# Autodesk Inventor assembly: Robot_Triciclo_(assembled_fixed)
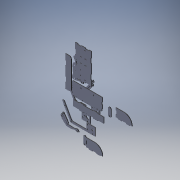
[picture p0: Inventor's stored thumbnail of the model, 180x180]
Saved by Autodesk Inventor 2019 (Build 230136000, 136)
## iProperties
Created: 2019-11-11
Part Number: Robot_Triciclo_(assembled_fixed)
Document SubType Name: Assembly
Designer: Domenico
Author: Domenico
Revision Number: ANY
## Documents named in this file (18)
- C:\Users\Domenico\Documents\Inventor\Mecanismos2\Robot_Triciclo_(assembled_fixed).iam
- C:\Users\Domenico\Documents\Inventor\Mecanismos2\Robot_Triciclo_(bike01).ipt
- C:\Users\Domenico\Documents\Inventor\Mecanismos2\Robot_Triciclo_(bike02).ipt
- C:\Users\Domenico\Documents\Inventor\Mecanismos2\Robot_Triciclo_(bike03).ipt
- C:\Users\Domenico\Documents\Inventor\Mecanismos2\Robot_Triciclo_(bike04).ipt
- C:\Users\Domenico\Documents\Inventor\Mecanismos2\Robot_Triciclo_(bike05).ipt
- C:\Users\Domenico\Documents\Inventor\Mecanismos2\Robot_Triciclo_(bike06).ipt
- C:\Users\Domenico\Documents\Inventor\Mecanismos2\Robot_Triciclo_(bike08).ipt
- C:\Users\Domenico\Documents\Inventor\Mecanismos2\Robot_Triciclo_(bike09).ipt
- C:\Users\Domenico\Documents\Inventor\Mecanismos2\Robot_Triciclo_(bike10).ipt
- C:\Users\Domenico\Documents\Inventor\Mecanismos2\Robot_Triciclo_(bike11).ipt
- C:\Users\Domenico\Documents\Inventor\Mecanismos2\Robot_Triciclo_(bike12).ipt
- C:\Users\Domenico\Documents\Inventor\Mecanismos2\Robot_Triciclo_(bike14).ipt
- C:\Users\Domenico\Documents\Inventor\Mecanismos2\Robot_Triciclo_(bike18).ipt
- C:\Users\Domenico\Documents\Inventor\Mecanismos2\Robot_Triciclo_(bike19).ipt
- C:\Users\Domenico\Documents\Inventor\Mecanismos2\Robot_Triciclo_(arms).ipt
- C:\Users\Domenico\Documents\Inventor\Mecanismos2\Robot_Triciclo_(body).ipt
- C:\Users\Domenico\Documents\Inventor\Mecanismos2\Robot_Triciclo_(head).ipt
## Components (23 placed, 23 different names)
1. Robot_Triciclo_(bike01)_54
2. Robot_Triciclo_(bike02)_55
3. Robot_Triciclo_(bike03)_56 — Mate:2, Mate:3
4. Robot_Triciclo_(bike04)_57 — Mate:2
5. Robot_Triciclo_(bike04)_58
6. Robot_Triciclo_(bike05)_59 — Mate:4
7. Robot_Triciclo_(bike06)_60 — Mate:3, Mate:4, Mate:5
8. Robot_Triciclo_(bike08)_61 — Mate:5
9. Robot_Triciclo_(bike09)_62
10. Robot_Triciclo_(bike09)_63
11. Robot_Triciclo_(bike10)_64 — Mate:1
12. Robot_Triciclo_(bike11)_65
13. Robot_Triciclo_(bike11)_66
14. Robot_Triciclo_(bike12)_67
15. Robot_Triciclo_(bike14)_68
16. Robot_Triciclo_(bike14)_69
17. Robot_Triciclo_(bike18)_70 — Mate:1
18. Robot_Triciclo_(bike19)_71
19. Robot_Triciclo_(bike19)_72
20. Robot_Triciclo_(arms)_73
21. Robot_Triciclo_(arms)_74
22. Robot_Triciclo_(body)_75
23. Robot_Triciclo_(head)_97
## Relationships (5: Mate 5)
- Mate:1: Robot_Triciclo_(bike10)_64 ↔ Robot_Triciclo_(bike18)_70
- Mate:2: Robot_Triciclo_(bike03)_56 ↔ Robot_Triciclo_(bike04)_57
- Mate:3: Robot_Triciclo_(bike03)_56 ↔ Robot_Triciclo_(bike06)_60
- Mate:4: Robot_Triciclo_(bike05)_59 ↔ Robot_Triciclo_(bike06)_60
- Mate:5: Robot_Triciclo_(bike06)_60 ↔ Robot_Triciclo_(bike08)_61
